# Autodesk Inventor assembly: drive with fourbar linkage
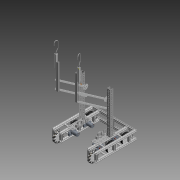
[picture p0: Inventor's stored thumbnail of the model, 180x180]
Saved by Autodesk Inventor 2013 (Build 170138000, 138)
## iProperties
Created: 2013-12-21
Part Number: drive with fourbar linkage
Document SubType Name: Assembly
Designer: kahohbein
Author: kahohbein
## Documents named in this file (14)
- C:\Users\kahohbein\Documents\GitHub\2013-2014_BlockParty\CAD\drive with fourbar linkage to bosch.iam
- C:\Users\kahohbein\Documents\GitHub\2013-2014_BlockParty\CAD\Drive\Final Drive Complete\Driveopen2.iam
- C:\Users\kahohbein\Documents\GitHub\2013-2014_BlockParty\CAD\COTSParts\Tetrix\Tetrix flat plate.ipt
- C:\Users\kahohbein\Documents\GitHub\2013-2014_BlockParty\CAD\COTSParts\Tetrix\Tetrix channel 32mm.ipt
- C:\Users\kahohbein\Documents\GitHub\2013-2014_BlockParty\CAD\COTSParts\Tetrix\Bronze bushing.ipt
- C:\Users\kahohbein\Documents\GitHub\2013-2014_BlockParty\CAD\COTSParts\Tetrix\Tetrix motor mount.ipt
- C:\Users\kahohbein\Documents\GitHub\2013-2014_BlockParty\CAD\Lift\MK3\hook prototype.ipt
- C:\Users\kahohbein\Documents\GitHub\2013-2014_BlockParty\CAD\Lift\Bosch 20x20 modified.ipt
- C:\Users\kahohbein\Documents\GitHub\2013-2014_BlockParty\CAD\four bar linkage\custom Box Aluminum.ipt
- C:\Users\kahohbein\Documents\GitHub\2013-2014_BlockParty\CAD\four bar linkage\custom bosch 8in.ipt
- C:\Users\kahohbein\Documents\GitHub\2013-2014_BlockParty\CAD\COTSParts\Tetrix\Tetrix Channel 416mm.ipt
- C:\Users\kahohbein\Documents\GitHub\2013-2014_BlockParty\CAD\COTSParts\Tetrix\Tetrix Channel 416mm_CPY.ipt
- C:\Users\kahohbein\Documents\GitHub\2013-2014_BlockParty\CAD\COTSParts\Tetrix\Tetrix Hub - axle.ipt
- C:\Users\kahohbein\Documents\GitHub\2013-2014_BlockParty\CAD\COTSParts\Tetrix\Tetrix sprocket 24T.ipt
## Components (27 placed, 13 different names)
1. Driveopen2:1 [sub-assembly] — Mate:1, Mate:2, Mate:3, Mate:4, Mate:5, Mate:6
2. Tetrix flat plate:1 — Mate:2, Mate:3, Mate:4, Mate:15, Mate:16, Mate:65, Mate:66, Mate:70, Mate:110, Flush:10
3. Tetrix flat plate:2 — Mate:1, Mate:5, Mate:6, Mate:11, Mate:12, Mate:67, Mate:68, Mate:69, Mate:100, Flush:8
4. Tetrix channel 32mm:1 — Mate:15, Mate:16, Flush:9, Mate:111, Flush:10
5. Tetrix channel 32mm:2 — Mate:11, Mate:12, Mate:101, Flush:7, Flush:8
6. Bronze bushing:6 — Mate:102, Mate:104
7. Bronze bushing:12 — Mate:103, Mate:105
8. Tetrix motor mount:1 — Mate:65, Mate:66, Mate:70
9. Tetrix motor mount:2 — Mate:67, Mate:68, Mate:69
10. hook prototype:1 — Mate:80, Mate:81
11. Bosch 20x20 modified:1 — Mate:80, Mate:81, Mate:99, Flush:6, Flush:11
12. custom Box Aluminum:1 — Flush:5, Mate:96, Mate:148, Mate:151, Mate:152
13. custom Box Aluminum:2 — Flush:4, Mate:97, Mate:98, Mate:140, Mate:143, Mate:144, Mate:145, Mate:146, Mate:147
14. custom Box Aluminum:3 — Flush:5, Mate:134, Mate:155, Mate:156
15. custom Box Aluminum:4 — Flush:4, Mate:124, Mate:126, Mate:129, Mate:130, Mate:131, Mate:135, Mate:136
16. custom bosch 8in:1 — Mate:96, Mate:97, Mate:98, Mate:99, Flush:6, Flush:11
17. Tetrix Channel 416mm:1 — Mate:100, Mate:101, Flush:7, Mate:102, Mate:103, Mate:104, Mate:105, Mate:140, Mate:141, Mate:142, Mate:148, Mate:149, Mate:150
18. Tetrix Channel 416mm_CPY:1 — Mate:110, Flush:9, Mate:111, Mate:132, Mate:133, Mate:153, Mate:154
19. Tetrix Hub - axle:1 — Mate:124, Mate:128, Mate:129, Mate:131, Mate:132, Mate:133
20. Tetrix sprocket 24T:1 — Mate:126, Mate:128, Mate:130
21. custom bosch 8in:2 — Mate:134, Mate:135, Mate:136, Mate:137, Flush:12, Flush:13
22. Bosch 20x20 modified:2 — Mate:137, Flush:12, Flush:13, Mate:138, Mate:139
23. hook prototype:2 — Mate:138, Mate:139
24. Tetrix Hub - axle:2 — Mate:141, Mate:142, Mate:143, Mate:144
25. Tetrix sprocket 24T:2 — Mate:145, Mate:146, Mate:147
26. Tetrix Hub - axle:3 — Mate:149, Mate:150, Mate:151, Mate:152
27. Tetrix Hub - axle:4 — Mate:153, Mate:154, Mate:155, Mate:156
## Relationships (71: Mate 61, Flush 10)
- Mate:1: Driveopen2:1 ↔ Tetrix flat plate:2
- Mate:2: Driveopen2:1 ↔ Tetrix flat plate:1
- Mate:3 (139.7 mm): Driveopen2:1 ↔ Tetrix flat plate:1
- Mate:4 (63.5 mm): Driveopen2:1 ↔ Tetrix flat plate:1
- Mate:5 (139.7 mm): Driveopen2:1 ↔ Tetrix flat plate:2
- Mate:6 (63.5 mm): Driveopen2:1 ↔ Tetrix flat plate:2
- Mate:11: Tetrix flat plate:2 ↔ Tetrix channel 32mm:2
- Mate:12: Tetrix flat plate:2 ↔ Tetrix channel 32mm:2
- Mate:15: Tetrix flat plate:1 ↔ Tetrix channel 32mm:1
- Mate:16: Tetrix flat plate:1 ↔ Tetrix channel 32mm:1
- Mate:65: Tetrix flat plate:1 ↔ Tetrix motor mount:1
- Mate:66: Tetrix flat plate:1 ↔ Tetrix motor mount:1
- Mate:67: Tetrix flat plate:2 ↔ Tetrix motor mount:2
- Mate:68: Tetrix flat plate:2 ↔ Tetrix motor mount:2
- Mate:69: Tetrix flat plate:2 ↔ Tetrix motor mount:2
- Mate:70: Tetrix flat plate:1 ↔ Tetrix motor mount:1
- Mate:80: hook prototype:1 ↔ Bosch 20x20 modified:1
- Mate:81: hook prototype:1 ↔ Bosch 20x20 modified:1
- Flush:4: custom Box Aluminum:2 ↔ custom Box Aluminum:4
- Flush:5: custom Box Aluminum:1 ↔ custom Box Aluminum:3
- Mate:96: custom Box Aluminum:1 ↔ custom bosch 8in:1
- Mate:97: custom Box Aluminum:2 ↔ custom bosch 8in:1
- Mate:98: custom Box Aluminum:2 ↔ custom bosch 8in:1
- Mate:99: Bosch 20x20 modified:1 ↔ custom bosch 8in:1
- Flush:6: Bosch 20x20 modified:1 ↔ custom bosch 8in:1
- Mate:100: Tetrix flat plate:2 ↔ Tetrix Channel 416mm:1
- Mate:101: Tetrix channel 32mm:2 ↔ Tetrix Channel 416mm:1
- Flush:7: Tetrix channel 32mm:2 ↔ Tetrix Channel 416mm:1
- Flush:8: Tetrix flat plate:2 ↔ Tetrix channel 32mm:2
- Mate:102: Bronze bushing:6 ↔ Tetrix Channel 416mm:1
- Mate:103: Bronze bushing:12 ↔ Tetrix Channel 416mm:1
- Mate:104: Bronze bushing:6 ↔ Tetrix Channel 416mm:1
- Mate:105: Bronze bushing:12 ↔ Tetrix Channel 416mm:1
- Mate:110: Tetrix flat plate:1 ↔ Tetrix Channel 416mm_CPY:1
- Flush:9: Tetrix channel 32mm:1 ↔ Tetrix Channel 416mm_CPY:1
- Mate:111: Tetrix channel 32mm:1 ↔ Tetrix Channel 416mm_CPY:1
- Flush:10: Tetrix flat plate:1 ↔ Tetrix channel 32mm:1
- Flush:11 (60.833 mm): Bosch 20x20 modified:1 ↔ custom bosch 8in:1
- Mate:124: custom Box Aluminum:4 ↔ Tetrix Hub - axle:1
- Mate:126: custom Box Aluminum:4 ↔ Tetrix sprocket 24T:1
- Mate:128: Tetrix Hub - axle:1 ↔ Tetrix sprocket 24T:1
- Mate:129: custom Box Aluminum:4 ↔ Tetrix Hub - axle:1
- Mate:130: custom Box Aluminum:4 ↔ Tetrix sprocket 24T:1
- Mate:131: custom Box Aluminum:4 ↔ Tetrix Hub - axle:1
- Mate:132: Tetrix Channel 416mm_CPY:1 ↔ Tetrix Hub - axle:1
- Mate:133: Tetrix Channel 416mm_CPY:1 ↔ Tetrix Hub - axle:1
- Mate:134: custom Box Aluminum:3 ↔ custom bosch 8in:2
- Mate:135: custom Box Aluminum:4 ↔ custom bosch 8in:2
- Mate:136: custom Box Aluminum:4 ↔ custom bosch 8in:2
- Mate:137: custom bosch 8in:2 ↔ Bosch 20x20 modified:2
- Flush:12: custom bosch 8in:2 ↔ Bosch 20x20 modified:2
- Flush:13 (-60.833 mm): custom bosch 8in:2 ↔ Bosch 20x20 modified:2
- Mate:138: Bosch 20x20 modified:2 ↔ hook prototype:2
- Mate:139 (-15.24 mm): Bosch 20x20 modified:2 ↔ hook prototype:2
- Mate:140: custom Box Aluminum:2 ↔ Tetrix Channel 416mm:1
- Mate:141: Tetrix Channel 416mm:1 ↔ Tetrix Hub - axle:2
- Mate:142: Tetrix Channel 416mm:1 ↔ Tetrix Hub - axle:2
- Mate:143: custom Box Aluminum:2 ↔ Tetrix Hub - axle:2
- Mate:144: custom Box Aluminum:2 ↔ Tetrix Hub - axle:2
- Mate:145: custom Box Aluminum:2 ↔ Tetrix sprocket 24T:2
- Mate:146: custom Box Aluminum:2 ↔ Tetrix sprocket 24T:2
- Mate:147: custom Box Aluminum:2 ↔ Tetrix sprocket 24T:2
- Mate:148: custom Box Aluminum:1 ↔ Tetrix Channel 416mm:1
- Mate:149: Tetrix Channel 416mm:1 ↔ Tetrix Hub - axle:3
- Mate:150: Tetrix Channel 416mm:1 ↔ Tetrix Hub - axle:3
- Mate:151: custom Box Aluminum:1 ↔ Tetrix Hub - axle:3
- Mate:152: custom Box Aluminum:1 ↔ Tetrix Hub - axle:3
- Mate:153: Tetrix Channel 416mm_CPY:1 ↔ Tetrix Hub - axle:4
- Mate:154: Tetrix Channel 416mm_CPY:1 ↔ Tetrix Hub - axle:4
- Mate:155: custom Box Aluminum:3 ↔ Tetrix Hub - axle:4
- Mate:156: custom Box Aluminum:3 ↔ Tetrix Hub - axle:4
